# Autodesk Inventor assembly: bellows_kihon
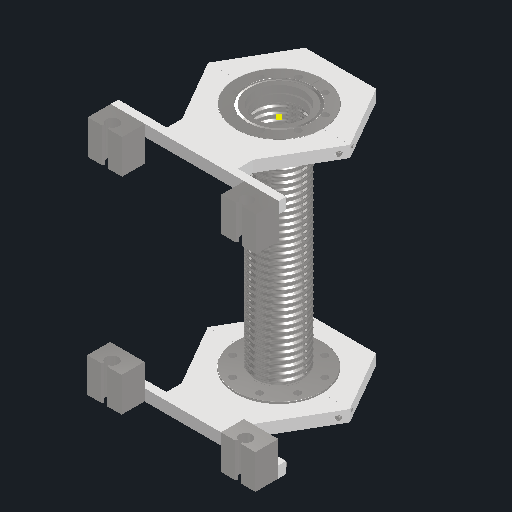
[picture p0: Inventor's stored thumbnail of the model, 512x512]
Saved by Autodesk Inventor 2026.3 (Build 303398000, 398)
## iProperties
Created: 2026-06-03
Part Number: bellows_kihon
Document SubType Name: Assembly
Designer: shusu
Author: shusu
## Documents named in this file (8)
- C:\Users\shusu\OneDrive - Kyoto University\デスクトップ\蓮尾研\ベローズ設計\bellows_kihon.iam
- C:\Users\shusu\OneDrive - Kyoto University\デスクトップ\蓮尾研\ベローズ設計\bellows_flange_2.ipt
- C:\Users\shusu\OneDrive - Kyoto University\デスクトップ\蓮尾研\ベローズ設計\bellows_bellows.ipt
- C:\Users\shusu\OneDrive - Kyoto University\デスクトップ\蓮尾研\ベローズ設計\nowtrying.ipt
- C:\Users\shusu\OneDrive - Kyoto University\デスクトップ\蓮尾研\ベローズ設計\nowtrying_up.ipt
- C:\Users\shusu\OneDrive - Kyoto University\ドキュメント\Inventor\Content Center Files\R2026\ja-JP\JIS B 1176\JIS B 1176 - M3 x 16 - 0.5.ipt
- C:\Users\shusu\OneDrive - Kyoto University\デスクトップ\蓮尾研\ベローズ設計\linearbearing.ipt
- C:\Users\shusu\OneDrive - Kyoto University\ドキュメント\Inventor\Content Center Files\R2026\ja-JP\JIS B 1176\JIS B 1176 - M5 x 16 - 0.8.ipt
## Components (23 placed, 7 different names)
1. bellows_flange_2:1 — 挿入:1, 角度:1, 挿入:3
2. bellows_bellows:1 — 挿入:1, 挿入:2
3. bellows_flange_2:2 — 挿入:2, 挿入:4
4. nowtrying:1 — メイト:1, メイト:2, 挿入:3, 挿入:9, 角度:2, メイト:5, メイト:7, 挿入:11, 挿入:12, 挿入:15, 挿入:16
5. nowtrying_up:1 — 角度:1, メイト:1, メイト:2, 挿入:7
6. nowtrying:3 — 挿入:4, 挿入:10, メイト:6, メイト:8, 挿入:13, 挿入:14, 挿入:17, 挿入:18
7. nowtrying_up:3 — 挿入:8
8. JIS B 1176 - メートル M3 x 16:3 — 挿入:7
9. JIS B 1176 - メートル M3 x 16:4 — 挿入:8
10. JIS B 1176 - メートル M3 x 16:5 — 挿入:9
11. JIS B 1176 - メートル M3 x 16:6 — 挿入:10
12. linearbearing:1 — 角度:2, メイト:5
13. linearbearing:2 — メイト:8
14. linearbearing:3 — メイト:6
15. linearbearing:4 — メイト:7
16. JIS B 1176 - メートル M5 x 16:1 — 挿入:11
17. JIS B 1176 - メートル M5 x 16:2 — 挿入:12
18. JIS B 1176 - メートル M5 x 16:3 — 挿入:13
19. JIS B 1176 - メートル M5 x 16:4 — 挿入:14
20. JIS B 1176 - メートル M5 x 16:5 — 挿入:15
21. JIS B 1176 - メートル M5 x 16:6 — 挿入:16
22. JIS B 1176 - メートル M5 x 16:7 — 挿入:18
23. JIS B 1176 - メートル M5 x 16:8 — 挿入:17
## Relationships (26: Insert 16, Mate 8, Angle 2)
- 挿入:1 [Insert] (-8 mm): bellows_flange_2:1 ↔ bellows_bellows:1
- 挿入:2 [Insert] (-8 mm): bellows_bellows:1 ↔ bellows_flange_2:2
- 角度:1 [Angle] (270 deg): bellows_flange_2:1 ↔ nowtrying_up:1
- メイト:1 [Mate]: nowtrying:1 ↔ nowtrying_up:1
- メイト:2 [Mate]: nowtrying:1 ↔ nowtrying_up:1
- [Mate]: nowtrying:3 ↔ nowtrying_up:3
- [Mate]: nowtrying:3 ↔ nowtrying_up:3
- 挿入:3 [Insert] (-15 mm): bellows_flange_2:1 ↔ nowtrying:1
- 挿入:4 [Insert] (-15 mm): bellows_flange_2:2 ↔ nowtrying:3
- 挿入:7 [Insert]: nowtrying_up:1 ↔ JIS B 1176 - メートル M3 x 16:3
- 挿入:8 [Insert]: nowtrying_up:3 ↔ JIS B 1176 - メートル M3 x 16:4
- 挿入:9 [Insert]: nowtrying:1 ↔ JIS B 1176 - メートル M3 x 16:5
- 挿入:10 [Insert]: nowtrying:3 ↔ JIS B 1176 - メートル M3 x 16:6
- 角度:2 [Angle] (0 deg): nowtrying:1 ↔ linearbearing:1
- メイト:5 [Mate]: nowtrying:1 ↔ linearbearing:1
- メイト:6 [Mate]: nowtrying:3 ↔ linearbearing:3
- メイト:7 [Mate]: nowtrying:1 ↔ linearbearing:4
- メイト:8 [Mate]: nowtrying:3 ↔ linearbearing:2
- 挿入:11 [Insert]: nowtrying:1 ↔ JIS B 1176 - メートル M5 x 16:1
- 挿入:12 [Insert]: nowtrying:1 ↔ JIS B 1176 - メートル M5 x 16:2
- 挿入:13 [Insert]: nowtrying:3 ↔ JIS B 1176 - メートル M5 x 16:3
- 挿入:14 [Insert]: nowtrying:3 ↔ JIS B 1176 - メートル M5 x 16:4
- 挿入:15 [Insert]: nowtrying:1 ↔ JIS B 1176 - メートル M5 x 16:5
- 挿入:16 [Insert]: nowtrying:1 ↔ JIS B 1176 - メートル M5 x 16:6
- 挿入:17 [Insert]: nowtrying:3 ↔ JIS B 1176 - メートル M5 x 16:8
- 挿入:18 [Insert]: nowtrying:3 ↔ JIS B 1176 - メートル M5 x 16:7
## Named parameters: d13_d11 = 0 mm, d14_d12 = 0 mm
